# Autodesk Inventor assembly: mirror_assembly_final
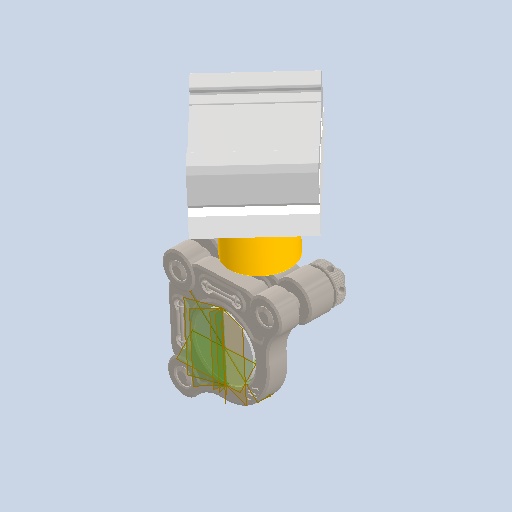
[picture p0: Inventor's stored thumbnail of the model, 512x512]
Saved by Autodesk Inventor 2026.1 (Build 301233000, 233)
## iProperties
Created: 2019-05-24
Part Number: mirror_assembly_final
Document SubType Name: Assembly
Designer: Julian
Author: Julian
## Documents named in this file (6)
- C:\Users\user\Desktop\setup for publishing\mirror_assembly_final - Kopie.iam
- C:\Users\user\Desktop\setup for publishing\XT66C2-Step_rail mount.ipt
- C:\Users\user\Desktop\setup for publishing\XT66D2-40-Step_post_mount.ipt
- C:\Users\user\Desktop\setup for publishing\M-PS-1E_1in_post.ipt
- C:\Users\user\Desktop\setup for publishing\SS100-F2H_suprema_1in_mirror_mount.ipt
- C:\Users\user\Desktop\setup for publishing\1in_5mm_mir.ipt
## Components (5 placed, 5 different names)
1. XT66C2-Step_rail mount:1 — Passend:5, Passend:6, Fluchtend:1, Winkel:1
2. XT66D2-40-Step_post_mount:1 — Passend:4, Passend:5, Passend:6, Fluchtend:1, Winkel:2
3. M-PS-1E_1in_post:1 — Passend:1, Passend:2, Passend:4
4. SS100-F2H_suprema_1in_mirror_mount:1 — Passend:1, Passend:2, Passend:7, Passend:8
5. 1in_5mm_mir:1 — Passend:7, Passend:8, Winkel:1, Winkel:2
## Relationships (10: Mate 7, Angle 2, Flush 1)
- Passend:1 [Mate]: M-PS-1E_1in_post:1 ↔ SS100-F2H_suprema_1in_mirror_mount:1
- Passend:2 [Mate]: M-PS-1E_1in_post:1 ↔ SS100-F2H_suprema_1in_mirror_mount:1
- Passend:4 [Mate]: XT66D2-40-Step_post_mount:1 ↔ M-PS-1E_1in_post:1
- Passend:5 [Mate]: XT66C2-Step_rail mount:1 ↔ XT66D2-40-Step_post_mount:1
- Passend:6 [Mate]: XT66C2-Step_rail mount:1 ↔ XT66D2-40-Step_post_mount:1
- Fluchtend:1 [Flush] (-0.0508 mm): XT66C2-Step_rail mount:1 ↔ XT66D2-40-Step_post_mount:1
- Passend:7 [Mate]: SS100-F2H_suprema_1in_mirror_mount:1 ↔ 1in_5mm_mir:1
- Passend:8 [Mate]: SS100-F2H_suprema_1in_mirror_mount:1 ↔ 1in_5mm_mir:1
- Winkel:1 [Angle] (225 deg): XT66C2-Step_rail mount:1 ↔ 1in_5mm_mir:1
- Winkel:2 [Angle] (0 deg): XT66D2-40-Step_post_mount:1 ↔ 1in_5mm_mir:1
